# Autodesk Inventor assembly: prototype4
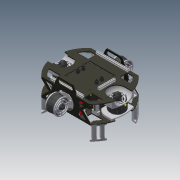
[picture p0: Inventor's stored thumbnail of the model, 180x180]
Saved by Autodesk Inventor 2018 (Build 220112000, 112)
## iProperties
Created: 2020-02-18
Part Number: prototype4
Document SubType Name: Assembly
Designer: anirudh
Author: anirudh
## Documents named in this file (32)
- D:\Silicon Sharks\2019-2020\prototype4\prototype4.iam
- D:\Silicon Sharks\2019-2020\prototype4\bottomPlate.ipt
- D:\Silicon Sharks\2019-2020\prototype4\sidePlate.ipt
- D:\Silicon Sharks\2019-2020\prototype4\topPlate.ipt
- D:\Silicon Sharks\2019-2020\prototype4\7inREV.ipt
- D:\Silicon Sharks\2019-2020\prototype4\handle.ipt
- D:\Silicon Sharks\2019-2020\ElectronicsHousing\Prototype2\ElectricalHousing2.iam
- D:\Silicon Sharks\2019-2020\prototype4\T200-THRUSTER.ipt
- D:\Silicon Sharks\2019-2020\prototype4\thrusterMounrt.ipt
- D:\Silicon Sharks\2019-2020\prototype4\4inREV.ipt
- D:\Silicon Sharks\2019-2020\prototype4\bottomThrusterCover.ipt
- D:\Silicon Sharks\2019-2020\prototype4\backSideThrusterCover.ipt
- D:\Silicon Sharks\2019-2020\prototype4\frontSideThrusterCover.ipt
- D:\Silicon Sharks\2019-2020\prototype4\topThrusterCover.ipt
- D:\Silicon Sharks\2019-2020\prototype4\acrylicMount.ipt
- D:\Silicon Sharks\2019-2020\prototype4\verticalAcrylicMount.ipt
- D:\Silicon Sharks\2019-2020\servoBox\servoAssembly.iam
- D:\Silicon Sharks\2019-2020\prototype4\bottomMountingPlate2.ipt
- D:\Silicon Sharks\2019-2020\prototype4\bottomCameraMount.ipt
- D:\Silicon Sharks\2019-2020\CameraEnclosure\CameraEnclosure1.iam
- D:\Silicon Sharks\2019-2020\prototype4\bottomCameraMount2.ipt
- D:\Silicon Sharks\2019-2020\prototype4\shaftMount.ipt
- D:\Silicon Sharks\2019-2020\servoBox\shaftSeal\6362K211_WATER-RESISTANT DRY-RUNNING SLEEVE BEARING.ipt
- D:\Silicon Sharks\2019-2020\prototype4\94868A004_18-8 SS FEM THRDED HEX STANDOFF.ipt
- D:\Silicon Sharks\2019-2020\clawGripper\bottomArms.ipt
- D:\Silicon Sharks\2019-2020\CameraEnclosure\cameraMount2.ipt
- D:\Silicon Sharks\2019-2020\CameraEnclosure\usbCamera.ipt
- D:\Silicon Sharks\2019-2020\clawGripper\bottomArms2.ipt
- D:\Silicon Sharks\2019-2020\clawGripper\topArm.ipt
- D:\Silicon Sharks\2019-2020\clawGripper\6462K190_SET SCREW SHAFT COLLAR (1).ipt
- D:\Silicon Sharks\2019-2020\prototype4\optimizedlandingGear v6.ipt
- D:\Silicon Sharks\2019-2020\prototype4\frameBracket.ipt
## Components (75 placed, 31 different names)
1. sidePlate:1 — Mate:17, Mate:47, Mate:48, Mate:49, Mate:257, Mate:259, Mate:260, Mate:261, Mate:263, Mate:264
2. sidePlate:2 — Mate:16, Mate:18, Mate:44, Mate:45, Mate:46, Flush:5, Mate:116, Mate:117, Mate:118, Mate:119, Mate:249, Mate:251, Mate:252, Mate:253, Mate:255, Mate:256
3. topPlate:2 — Mate:16, Mate:17, Mate:18, Mate:19, Flush:1, Mate:20, Mate:21, Mate:22, Flush:2, Mate:24, Mate:26, Mate:28, Mate:56, Mate:57, Mate:58, Mate:77, Mate:78, Mate:79, Mate:91, Mate:92, Mate:93, Mate:119, Mate:214, Mate:215, Flush:202, Mate:216, Mate:217, Flush:203, Mate:250, Mate:254
4. 7inREV:1 — Mate:19, Flush:1, Mate:20, Mate:27
5. 7inREV:2 — Mate:21, Mate:22, Flush:2, Mate:23, Mate:25
6. handle:1 — Mate:26, Mate:27, Mate:28
7. handle:2 — Mate:23, Mate:24, Mate:25
8. ElectricalHousing2:1 [sub-assembly]
9. T200-THRUSTER:1
10. T200-THRUSTER:2 — Mate:101
11. thrusterMounrt:1 — Mate:44, Mate:45, Mate:46, Mate:50, Mate:51, Mate:52, Mate:71, Mate:110, Mate:265
12. thrusterMounrt:2 — Mate:47, Mate:48, Mate:49, Mate:53, Mate:54, Mate:55, Mate:74, Mate:113, Mate:266
13. T200-THRUSTER:3 — Mate:50, Mate:51, Mate:52, Flush:3, Mate:73, Flush:7
14. T200-THRUSTER:4 — Mate:53, Mate:54, Mate:55, Mate:76
15. 4inREV:1 — Mate:56, Mate:57, Mate:58
16. bottomThrusterCover:1
17. bottomThrusterCover:2
18. backSideThrusterCover:1 — Mate:110, Mate:265
19. backSideThrusterCover:2 — Mate:113, Mate:266
20. frontSideThrusterCover:1 — Mate:71, Mate:72, Mate:73
21. frontSideThrusterCover:2 — Mate:74, Mate:75, Mate:76
22. topThrusterCover:1 — Mate:77, Mate:78, Mate:79
23. acrylicMount:1 — Mate:88
24. acrylicMount:2 — Mate:89, Mate:90
25. verticalAcrylicMount:1 — Mate:88, Mate:89, Mate:90
26. topThrusterCover:2 — Mate:91, Mate:92, Mate:93
27. acrylicMount:3 — Mate:102, Mate:103
28. acrylicMount:4 — Mate:100
29. verticalAcrylicMount:2 — Mate:100, Mate:101, Mate:102, Mate:103
30. servoAssembly:1 [sub-assembly] — Mate:124, Mate:125, Mate:126, Mate:240, Mate:241, Mate:242, Mate:243, Mate:244, Mate:245, Mate:246, Mate:247, Mate:248
31. bottomPlate:1 — Mate:116, Mate:117, Mate:118, Mate:120, Mate:121, Mate:122, Mate:123, Mate:124, Mate:125, Mate:126, Flush:10, Mate:169, Mate:170, Mate:171, Mate:180, Mate:181, Mate:182, Mate:228, Mate:229, Mate:230, Mate:231, Mate:232, Mate:233, Mate:234, Mate:235, Mate:236, Mate:237, Mate:238, Mate:239, Mate:258, Mate:262
32. bottomMountingPlate2:1 — Mate:140, Mate:141, Mate:142, Mate:143, Mate:144, Mate:145, Mate:172, Mate:173, Mate:174, Mate:175, Mate:176, Mate:177, Mate:178, Mate:179, Mate:183, Mate:184, Mate:185
33. bottomCameraMount:1 — Mate:140, Mate:141, Mate:142, Mate:146, Mate:148, Flush:8, Symmetry:3
34. bottomCameraMount:2 — Mate:143, Mate:144, Mate:145, Mate:147, Mate:150, Flush:9, Symmetry:3
35. CameraEnclosure1:1 [sub-assembly] — Mate:146, Mate:147, Mate:149, Mate:151, Mate:186
36. bottomCameraMount2:1 — Mate:148, Mate:149, Flush:8
37. bottomCameraMount2:2 — Mate:150, Mate:151, Flush:9
38. shaftMount:1 — Mate:165, Mate:167, Mate:169, Mate:170, Mate:171
39. 6362K211_WATER-RESISTANT DRY-RUNNING SLEEVE BEARING:1 — Mate:167, Mate:241
40. 6362K211_WATER-RESISTANT DRY-RUNNING SLEEVE BEARING:2 — Mate:165, Mate:240
41. 94868A004_18-8 SS FEM THRDED HEX STANDOFF:1 — Mate:174, Mate:175
42. 94868A004_18-8 SS FEM THRDED HEX STANDOFF:2 — Mate:178, Mate:179, Mate:180, Mate:182
43. 94868A004_18-8 SS FEM THRDED HEX STANDOFF:3 — Mate:176, Mate:177, Mate:181
44. 94868A004_18-8 SS FEM THRDED HEX STANDOFF:4 — Mate:172, Mate:173
45. bottomArms:1 — Mate:183, Mate:184, Mate:185, Mate:191, Mate:192, Mate:193, Mate:194, Mate:195, Mate:196
46. cameraMount2:1 — Mate:188, Flush:15, Flush:16, Symmetry:1, Symmetry:2
47. cameraMount2:2 — Mate:187, Flush:13, Flush:14, Symmetry:1, Symmetry:2, Mate:189
48. usbCamera:1 — Mate:187, Flush:13, Flush:14, Mate:188, Flush:15, Flush:16
49. bottomArms2:1 — Mate:194, Mate:195, Mate:196, Symmetry:4, Mate:204
50. bottomArms2:2 — Mate:191, Mate:192, Mate:193, Symmetry:4, Mate:202
51. topArm:1 — Mate:197, Flush:199, Mate:198, Mate:200, Flush:200, Flush:201
52. 6462K190_SET SCREW SHAFT COLLAR (1):1 — Mate:208, Mate:247
53. 6462K190_SET SCREW SHAFT COLLAR (1):2 — Mate:206, Mate:248
54. 6462K190_SET SCREW SHAFT COLLAR (1):3 — Mate:210, Mate:244
55. 6462K190_SET SCREW SHAFT COLLAR (1):4 — Mate:212, Mate:243
56. 6462K190_SET SCREW SHAFT COLLAR (1):5 — Mate:200, Mate:245
57. 6462K190_SET SCREW SHAFT COLLAR (1):6 — Mate:198, Mate:246
58. topArm:2 — Mate:202, Flush:200, Mate:206, Mate:208
59. topArm:3 — Mate:204, Flush:201, Mate:210, Mate:212, Mate:242
60. bottomCameraMount:3 — Mate:216, Mate:217, Flush:203, Mate:219, Mate:222, Flush:205, Symmetry:5
61. bottomCameraMount2:3 — Mate:220, Flush:204, Mate:221
62. bottomCameraMount:4 — Mate:214, Mate:215, Flush:202, Mate:218, Mate:220, Flush:204, Symmetry:5
63. bottomCameraMount2:4 — Mate:222, Flush:205, Mate:223
64. CameraEnclosure1:2 [sub-assembly] — Mate:218, Mate:219, Mate:221, Mate:223, Mate:226
65. cameraMount2:3 — Mate:224, Flush:206, Flush:207, Symmetry:6, Mate:226
66. cameraMount2:4 — Mate:225, Flush:208, Flush:209, Symmetry:6
67. usbCamera:2 — Mate:224, Flush:206, Flush:207, Mate:225, Flush:208, Flush:209
68. optimizedlandingGear v6:1 — Mate:228, Mate:229, Mate:230
69. optimizedlandingGear v6:2 — Mate:231, Mate:232, Mate:233
70. optimizedlandingGear v6:3 — Mate:234, Mate:238, Mate:239
71. optimizedlandingGear v6:4 — Mate:235, Mate:236, Mate:237
72. frameBracket:1 — Mate:249, Mate:250, Mate:251, Mate:252
73. frameBracket:2 — Mate:253, Mate:254, Mate:255, Mate:256
74. frameBracket:3 — Mate:257, Mate:258, Mate:259, Mate:260
75. frameBracket:4 — Mate:261, Mate:262, Mate:263, Mate:264
## Relationships (195: Mate 164, Flush 25, Symmetry 6)
- Mate:16: sidePlate:2 ↔ topPlate:2
- Mate:17: sidePlate:1 ↔ topPlate:2
- Mate:18: sidePlate:2 ↔ topPlate:2
- Mate:19: topPlate:2 ↔ 7inREV:1
- Flush:1 (5.588 mm): topPlate:2 ↔ 7inREV:1
- Mate:20: topPlate:2 ↔ 7inREV:1
- Mate:21: topPlate:2 ↔ 7inREV:2
- Mate:22: topPlate:2 ↔ 7inREV:2
- Flush:2 (5.588 mm): topPlate:2 ↔ 7inREV:2
- Mate:23: 7inREV:2 ↔ handle:2
- Mate:24: topPlate:2 ↔ handle:2
- Mate:25: 7inREV:2 ↔ handle:2
- Mate:26: topPlate:2 ↔ handle:1
- Mate:27: 7inREV:1 ↔ handle:1
- Mate:28: topPlate:2 ↔ handle:1
- Mate:44: sidePlate:2 ↔ thrusterMounrt:1
- Mate:45: sidePlate:2 ↔ thrusterMounrt:1
- Mate:46: sidePlate:2 ↔ thrusterMounrt:1
- Mate:47: sidePlate:1 ↔ thrusterMounrt:2
- Mate:48: sidePlate:1 ↔ thrusterMounrt:2
- Mate:49: sidePlate:1 ↔ thrusterMounrt:2
- Mate:50: thrusterMounrt:1 ↔ T200-THRUSTER:3
- Mate:51: thrusterMounrt:1 ↔ T200-THRUSTER:3
- Mate:52: thrusterMounrt:1 ↔ T200-THRUSTER:3
- Mate:53: thrusterMounrt:2 ↔ T200-THRUSTER:4
- Mate:54: thrusterMounrt:2 ↔ T200-THRUSTER:4
- Mate:55: thrusterMounrt:2 ↔ T200-THRUSTER:4
- Mate:56: topPlate:2 ↔ 4inREV:1
- Mate:57: topPlate:2 ↔ 4inREV:1
- Mate:58: topPlate:2 ↔ 4inREV:1
- Flush:3: T200-THRUSTER:3
- Flush:4 (-12.7 mm)
- Flush:5: sidePlate:2
- Flush:6 (-119.7864 mm)
- Mate:71: thrusterMounrt:1 ↔ frontSideThrusterCover:1
- Mate:72: frontSideThrusterCover:1
- Mate:73: T200-THRUSTER:3 ↔ frontSideThrusterCover:1
- Mate:74: thrusterMounrt:2 ↔ frontSideThrusterCover:2
- Mate:75: frontSideThrusterCover:2
- Mate:76: T200-THRUSTER:4 ↔ frontSideThrusterCover:2
- Mate:77: topPlate:2 ↔ topThrusterCover:1
- Mate:78: topPlate:2 ↔ topThrusterCover:1
- Mate:79: topPlate:2 ↔ topThrusterCover:1
- Mate:88: acrylicMount:1 ↔ verticalAcrylicMount:1
- Mate:89: acrylicMount:2 ↔ verticalAcrylicMount:1
- Mate:90: acrylicMount:2 ↔ verticalAcrylicMount:1
- Mate:91: topPlate:2 ↔ topThrusterCover:2
- Mate:92: topPlate:2 ↔ topThrusterCover:2
- Mate:93: topPlate:2 ↔ topThrusterCover:2
- Mate:100: acrylicMount:4 ↔ verticalAcrylicMount:2
- Mate:101: T200-THRUSTER:2 ↔ verticalAcrylicMount:2
- Mate:102: acrylicMount:3 ↔ verticalAcrylicMount:2
- Mate:103: acrylicMount:3 ↔ verticalAcrylicMount:2
- Flush:7 (-17.78 mm): T200-THRUSTER:3
- Mate:110: thrusterMounrt:1 ↔ backSideThrusterCover:1
- Mate:113: thrusterMounrt:2 ↔ backSideThrusterCover:2
- Mate:116: sidePlate:2 ↔ bottomPlate:1
- Mate:117: sidePlate:2 ↔ bottomPlate:1
- Mate:118: sidePlate:2 ↔ bottomPlate:1
- Mate:119: sidePlate:2 ↔ topPlate:2
- Mate:120: bottomPlate:1
- Mate:121: bottomPlate:1
- Mate:122: bottomPlate:1
- Mate:123: bottomPlate:1
- Mate:124: servoAssembly:1 ↔ bottomPlate:1
- Mate:125: servoAssembly:1 ↔ bottomPlate:1
- Mate:126: servoAssembly:1 ↔ bottomPlate:1
- Mate:140: bottomMountingPlate2:1 ↔ bottomCameraMount:1
- Mate:141: bottomMountingPlate2:1 ↔ bottomCameraMount:1
- Mate:142: bottomMountingPlate2:1 ↔ bottomCameraMount:1
- Mate:143: bottomMountingPlate2:1 ↔ bottomCameraMount:2
- Mate:144: bottomMountingPlate2:1 ↔ bottomCameraMount:2
- Mate:145: bottomMountingPlate2:1 ↔ bottomCameraMount:2
- Mate:146: bottomCameraMount:1 ↔ CameraEnclosure1:1
- Mate:147 (0.0381 mm): bottomCameraMount:2 ↔ CameraEnclosure1:1
- Mate:148: bottomCameraMount:1 ↔ bottomCameraMount2:1
- Mate:149: CameraEnclosure1:1 ↔ bottomCameraMount2:1
- Flush:8: bottomCameraMount:1 ↔ bottomCameraMount2:1
- Mate:150: bottomCameraMount:2 ↔ bottomCameraMount2:2
- Mate:151: CameraEnclosure1:1 ↔ bottomCameraMount2:2
- Flush:9: bottomCameraMount:2 ↔ bottomCameraMount2:2
- Flush:10 (88.9 mm): bottomPlate:1
- Mate:165: shaftMount:1 ↔ 6362K211_WATER-RESISTANT DRY-RUNNING SLEEVE BEARING:2
- Mate:167: shaftMount:1 ↔ 6362K211_WATER-RESISTANT DRY-RUNNING SLEEVE BEARING:1
- Mate:169: bottomPlate:1 ↔ shaftMount:1
- Mate:170: bottomPlate:1 ↔ shaftMount:1
- Mate:171: bottomPlate:1 ↔ shaftMount:1
- Mate:172: bottomMountingPlate2:1 ↔ 94868A004_18-8 SS FEM THRDED HEX STANDOFF:4
- Mate:173: bottomMountingPlate2:1 ↔ 94868A004_18-8 SS FEM THRDED HEX STANDOFF:4
- Mate:174: bottomMountingPlate2:1 ↔ 94868A004_18-8 SS FEM THRDED HEX STANDOFF:1
- Mate:175: bottomMountingPlate2:1 ↔ 94868A004_18-8 SS FEM THRDED HEX STANDOFF:1
- Mate:176: bottomMountingPlate2:1 ↔ 94868A004_18-8 SS FEM THRDED HEX STANDOFF:3
- Mate:177: bottomMountingPlate2:1 ↔ 94868A004_18-8 SS FEM THRDED HEX STANDOFF:3
- Mate:178: bottomMountingPlate2:1 ↔ 94868A004_18-8 SS FEM THRDED HEX STANDOFF:2
- Mate:179: bottomMountingPlate2:1 ↔ 94868A004_18-8 SS FEM THRDED HEX STANDOFF:2
- Mate:180: bottomPlate:1 ↔ 94868A004_18-8 SS FEM THRDED HEX STANDOFF:2
- Mate:181: bottomPlate:1 ↔ 94868A004_18-8 SS FEM THRDED HEX STANDOFF:3
- Mate:182: bottomPlate:1 ↔ 94868A004_18-8 SS FEM THRDED HEX STANDOFF:2
- Mate:183: bottomMountingPlate2:1 ↔ bottomArms:1
- Mate:184: bottomMountingPlate2:1 ↔ bottomArms:1
- Mate:185: bottomMountingPlate2:1 ↔ bottomArms:1
- Mate:186: CameraEnclosure1:1
- Mate:187: cameraMount2:2 ↔ usbCamera:1
- Flush:13 (-2.0066 mm): cameraMount2:2 ↔ usbCamera:1
- Flush:14 (2.0574 mm): cameraMount2:2 ↔ usbCamera:1
- Mate:188: cameraMount2:1 ↔ usbCamera:1
- Flush:15 (-2.0574 mm): cameraMount2:1 ↔ usbCamera:1
- Flush:16 (-2.0066 mm): cameraMount2:1 ↔ usbCamera:1
- Symmetry:1: cameraMount2:1 ↔ cameraMount2:2
- Symmetry:2: cameraMount2:1 ↔ cameraMount2:2
- Mate:189: cameraMount2:2
- Symmetry:3: bottomCameraMount:1 ↔ bottomCameraMount:2
- Mate:190
- Mate:191: bottomArms:1 ↔ bottomArms2:2
- Mate:192: bottomArms:1 ↔ bottomArms2:2
- Mate:193: bottomArms:1 ↔ bottomArms2:2
- Mate:194: bottomArms:1 ↔ bottomArms2:1
- Mate:195: bottomArms:1 ↔ bottomArms2:1
- Mate:196: bottomArms:1 ↔ bottomArms2:1
- Symmetry:4: bottomArms2:1 ↔ bottomArms2:2
- Mate:197: topArm:1
- Flush:199: topArm:1
- Mate:198: topArm:1 ↔ 6462K190_SET SCREW SHAFT COLLAR (1):6
- Mate:200: topArm:1 ↔ 6462K190_SET SCREW SHAFT COLLAR (1):5
- Mate:202 (3.556 mm): bottomArms2:2 ↔ topArm:2
- Flush:200: topArm:1 ↔ topArm:2
- Mate:204 (3.556 mm): bottomArms2:1 ↔ topArm:3
- Flush:201: topArm:1 ↔ topArm:3
- Mate:206: 6462K190_SET SCREW SHAFT COLLAR (1):2 ↔ topArm:2
- Mate:208: 6462K190_SET SCREW SHAFT COLLAR (1):1 ↔ topArm:2
- Mate:210: 6462K190_SET SCREW SHAFT COLLAR (1):3 ↔ topArm:3
- Mate:212: 6462K190_SET SCREW SHAFT COLLAR (1):4 ↔ topArm:3
- Mate:214: topPlate:2 ↔ bottomCameraMount:4
- Mate:215: topPlate:2 ↔ bottomCameraMount:4
- Flush:202: topPlate:2 ↔ bottomCameraMount:4
- Mate:216: topPlate:2 ↔ bottomCameraMount:3
- Mate:217: topPlate:2 ↔ bottomCameraMount:3
- Flush:203: topPlate:2 ↔ bottomCameraMount:3
- Mate:218: bottomCameraMount:4 ↔ CameraEnclosure1:2
- Mate:219 (0.0381 mm): bottomCameraMount:3 ↔ CameraEnclosure1:2
- Mate:220: bottomCameraMount2:3 ↔ bottomCameraMount:4
- Flush:204: bottomCameraMount2:3 ↔ bottomCameraMount:4
- Mate:221: bottomCameraMount2:3 ↔ CameraEnclosure1:2
- Mate:222: bottomCameraMount:3 ↔ bottomCameraMount2:4
- Flush:205: bottomCameraMount:3 ↔ bottomCameraMount2:4
- Mate:223: bottomCameraMount2:4 ↔ CameraEnclosure1:2
- Mate:224: cameraMount2:3 ↔ usbCamera:2
- Flush:206 (-2.0066 mm): cameraMount2:3 ↔ usbCamera:2
- Flush:207 (-2.0574 mm): cameraMount2:3 ↔ usbCamera:2
- Mate:225: cameraMount2:4 ↔ usbCamera:2
- Flush:208 (-2.0574 mm): cameraMount2:4 ↔ usbCamera:2
- Flush:209 (-2.0066 mm): cameraMount2:4 ↔ usbCamera:2
- Symmetry:5: bottomCameraMount:3 ↔ bottomCameraMount:4
- Symmetry:6: cameraMount2:3 ↔ cameraMount2:4
- Mate:226: CameraEnclosure1:2 ↔ cameraMount2:3
- Mate:227
- Mate:228: bottomPlate:1 ↔ optimizedlandingGear v6:1
- Mate:229: bottomPlate:1 ↔ optimizedlandingGear v6:1
- Mate:230: bottomPlate:1 ↔ optimizedlandingGear v6:1
- Mate:231: bottomPlate:1 ↔ optimizedlandingGear v6:2
- Mate:232: bottomPlate:1 ↔ optimizedlandingGear v6:2
- Mate:233: bottomPlate:1 ↔ optimizedlandingGear v6:2
- Mate:234: bottomPlate:1 ↔ optimizedlandingGear v6:3
- Mate:235: bottomPlate:1 ↔ optimizedlandingGear v6:4
- Mate:236: bottomPlate:1 ↔ optimizedlandingGear v6:4
- Mate:237: bottomPlate:1 ↔ optimizedlandingGear v6:4
- Mate:238: bottomPlate:1 ↔ optimizedlandingGear v6:3
- Mate:239: bottomPlate:1 ↔ optimizedlandingGear v6:3
- Mate:240: servoAssembly:1 ↔ 6362K211_WATER-RESISTANT DRY-RUNNING SLEEVE BEARING:2
- Mate:241: servoAssembly:1 ↔ 6362K211_WATER-RESISTANT DRY-RUNNING SLEEVE BEARING:1
- Mate:242: servoAssembly:1 ↔ topArm:3
- Mate:243: servoAssembly:1 ↔ 6462K190_SET SCREW SHAFT COLLAR (1):4
- Mate:244: servoAssembly:1 ↔ 6462K190_SET SCREW SHAFT COLLAR (1):3
- Mate:245: servoAssembly:1 ↔ 6462K190_SET SCREW SHAFT COLLAR (1):5
- Mate:246: servoAssembly:1 ↔ 6462K190_SET SCREW SHAFT COLLAR (1):6
- Mate:247: servoAssembly:1 ↔ 6462K190_SET SCREW SHAFT COLLAR (1):1
- Mate:248: servoAssembly:1 ↔ 6462K190_SET SCREW SHAFT COLLAR (1):2
- Mate:249: sidePlate:2 ↔ frameBracket:1
- Mate:250: topPlate:2 ↔ frameBracket:1
- Mate:251: sidePlate:2 ↔ frameBracket:1
- Mate:252: sidePlate:2 ↔ frameBracket:1
- Mate:253: sidePlate:2 ↔ frameBracket:2
- Mate:254: topPlate:2 ↔ frameBracket:2
- Mate:255: sidePlate:2 ↔ frameBracket:2
- Mate:256: sidePlate:2 ↔ frameBracket:2
- Mate:257: sidePlate:1 ↔ frameBracket:3
- Mate:258: bottomPlate:1 ↔ frameBracket:3
- Mate:259: sidePlate:1 ↔ frameBracket:3
- Mate:260: sidePlate:1 ↔ frameBracket:3
- Mate:261: sidePlate:1 ↔ frameBracket:4
- Mate:262: bottomPlate:1 ↔ frameBracket:4
- Mate:263: sidePlate:1 ↔ frameBracket:4
- Mate:264: sidePlate:1 ↔ frameBracket:4
- Mate:265: thrusterMounrt:1 ↔ backSideThrusterCover:1
- Mate:266: thrusterMounrt:2 ↔ backSideThrusterCover:2
